# Autodesk Inventor assembly: 275-1272
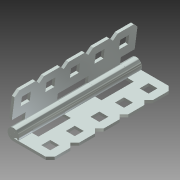
[picture p0: Inventor's stored thumbnail of the model, 180x180]
Saved by Autodesk Inventor 2013 (Build 170138000, 138)
## iProperties
Category: Structure
Company: Autodesk Inc.
Created: 2012-02-08
Part Number: 275-1272
Document SubType Name: Assembly
Designer: Autodesk Inc.
Catalog Web Link: http://www.vexrobotics.com/products/accessories/structure/275-1272.html
Vendor: VEX
Author: Autodesk Inc.
## Documents named in this file (4)
- C:\Data Folder\VEX 2012\VEX KOP Uploads\2013\Imperial\Structure\Hinge.iam
- C:\Data Folder\VEX 2012\VEX KOP Uploads\2013\Imperial\Structure\Components\VEX-HINGE-1 RevA.ipt
- C:\Data Folder\VEX 2012\VEX KOP Uploads\2013\Imperial\Structure\Components\VEX-HINGE-2 RevA.ipt
- C:\Data Folder\VEX 2012\VEX KOP Uploads\2013\Imperial\Structure\Components\VEX-HINGE-PIN.ipt
## Components (3 placed, 3 different names)
1. VEX-HINGE-1 RevA:1 — Insert:1, Insert:2
2. VEX-HINGE-2 RevA:1 — Insert:1
3. VEX-HINGE-PIN:1 — Insert:2
## Relationships (2: Insert 2)
- Insert:1: VEX-HINGE-1 RevA:1 ↔ VEX-HINGE-2 RevA:1
- Insert:2: VEX-HINGE-1 RevA:1 ↔ VEX-HINGE-PIN:1
